# Autodesk Inventor assembly: A1200KBv2
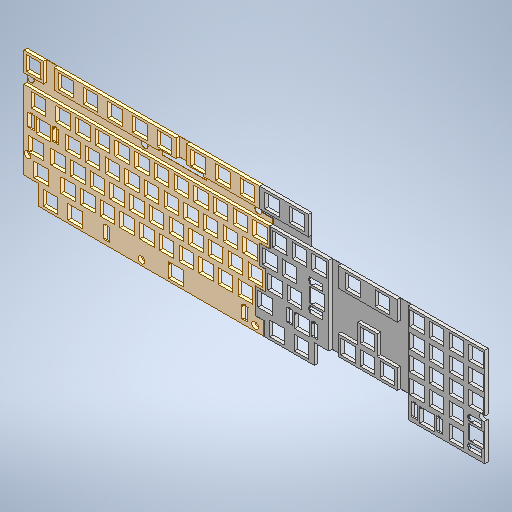
[picture p0: Inventor's stored thumbnail of the model, 512x512]
Saved by Autodesk Inventor 2025 (Build 290162000, 162)
## iProperties
Created: 2024-07-10
Part Number: A1200KBv2
Document SubType Name: Assembly
Designer: adam
Author: adam
## Documents named in this file (4)
- C:\Users\adam\Projects\A1200KBv2\3dprint\Keyboard plates\A1200KBv2.iam
- C:\Users\adam\Projects\A1200KBv2\3dprint\Keyboard plates\PCB.ipt
- C:\Users\adam\Projects\A1200KBv2\3dprint\Keyboard plates\Left Plate.ipt
- C:\Users\adam\Projects\A1200KBv2\3dprint\Keyboard plates\Right Plate.ipt
## Components (3 placed, 3 different names)
1. PCB:1 — Flush:1, Flush:2
2. Left Plate:1 — Flush:1
3. Right Plate:1 — Flush:2
## Relationships (2: Flush 2)
- Flush:1: PCB:1 ↔ Left Plate:1
- Flush:2: PCB:1 ↔ Right Plate:1
